# Autodesk Inventor assembly: +XPanel
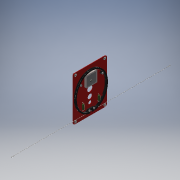
[picture p0: Inventor's stored thumbnail of the model, 180x180]
Saved by Autodesk Inventor 2018 (Build 220112000, 112)
## iProperties
Created: 2018-07-05
Part Number: +XPanel
Document SubType Name: Assembly
Designer: Bradley
Mass: 19.8214 g
Surface Area: 182.188 cm^2
Volume: 10.2774 cm^3
Density: 1.92865 g/cm^3
Author: Bradley
## Documents named in this file (10)
- D:\Users\Bradley\Documents\CougsInSpace\CougSat1-Hardware\CougSat1-AvionicBoard\CADModel\Native\+XPanel.iam
- D:\Users\Bradley\Documents\CougsInSpace\CougSat1-Hardware\CougSat1-AvionicBoard\CADModel\Native\+XPanel_PCB.ipt
- D:\Users\Bradley\Documents\CougsInSpace\Resources\ComponentModels\Electronics\Antenna_GPSPatch.ipt
- D:\Users\Bradley\Documents\CougsInSpace\Resources\ComponentModels\Fasteners\Bolt_M3x0.35_5mm_BH.ipt
- D:\Users\Bradley\Documents\CougsInSpace\CougSat1-Hardware\CougSat1-AvionicBoard\CADModel\Native\+XPanel_AntennaDeployed.ipt
- D:\Users\Bradley\Documents\CougsInSpace\CougSat1-Hardware\CougSat1-AvionicBoard\CADModel\Native\+XPanel_AntennaMount.ipt
- D:\Users\Bradley\Documents\CougsInSpace\CougSat1-Hardware\CougSat1-AvionicBoard\CADModel\Native\+XPanel_AntennaForm.ipt
- D:\Users\Bradley\Documents\CougsInSpace\Resources\ComponentModels\Fasteners\Bolt_M2x0.4_6mm_SH.ipt
- D:\Users\Bradley\Documents\CougsInSpace\CougSat1-Hardware\CougSat1-AvionicBoard\CADModel\Native\+XPanel_AntennaStowed+Y.ipt
- D:\Users\Bradley\Documents\CougsInSpace\Resources\ComponentModels\Electronics\Resistor_TH-15mm.ipt
## Components (17 placed, 9 different names)
1. +XPanel_PCB:1 — Insert:1, Insert:2, Insert:3, Insert:4, Insert:5, Mate:2, Mate:3, Insert:10, Insert:11, Insert:14, Insert:15, Insert:20, Insert:21, Insert:22, Insert:23
2. Antenna_GPSPatch:1 — Flush:1, Insert:1
3. Bolt_M3x0.35_5mm_BH:1 — Insert:2
4. Bolt_M3x0.35_5mm_BH:2 — Insert:3
5. Bolt_M3x0.35_5mm_BH:3 — Insert:4
6. Bolt_M3x0.35_5mm_BH:4 — Insert:5
7. +XPanel_AntennaDeployed:1 — Mate:1, Mate:2, Flush:2
8. +XPanel_AntennaDeployed:2 — Mate:3, Mate:4
9. +XPanel_AntennaMount:1 — Mate:1, Mate:4, Insert:16, Insert:17, Insert:18, Insert:19
10. +XPanel_AntennaForm:1 — Insert:10, Insert:11, Insert:12, Insert:13, Insert:14, Insert:15, Insert:16, Insert:17, Mate:5
11. Bolt_M2x0.4_6mm_SH:1 — Insert:12
12. Bolt_M2x0.4_6mm_SH:2 — Insert:13
13. Bolt_M2x0.4_6mm_SH:3 — Insert:19
14. Bolt_M2x0.4_6mm_SH:4 — Insert:18
15. +XPanel_AntennaStowed+Y:1 — Mate:5, Flush:2
16. Resistor_TH-15mm:1 — Insert:20, Insert:21
17. Resistor_TH-15mm:2 — Insert:22, Insert:23
## Relationships (26: Insert 19, Mate 5, Flush 2)
- Flush:1: Antenna_GPSPatch:1
- Insert:1: +XPanel_PCB:1 ↔ Antenna_GPSPatch:1
- Insert:2: +XPanel_PCB:1 ↔ Bolt_M3x0.35_5mm_BH:1
- Insert:3: +XPanel_PCB:1 ↔ Bolt_M3x0.35_5mm_BH:2
- Insert:4: +XPanel_PCB:1 ↔ Bolt_M3x0.35_5mm_BH:3
- Insert:5: +XPanel_PCB:1 ↔ Bolt_M3x0.35_5mm_BH:4
- Mate:1: +XPanel_AntennaDeployed:1 ↔ +XPanel_AntennaMount:1
- Mate:2: +XPanel_PCB:1 ↔ +XPanel_AntennaDeployed:1
- Mate:3: +XPanel_PCB:1 ↔ +XPanel_AntennaDeployed:2
- Mate:4: +XPanel_AntennaDeployed:2 ↔ +XPanel_AntennaMount:1
- Insert:10: +XPanel_PCB:1 ↔ +XPanel_AntennaForm:1
- Insert:11: +XPanel_PCB:1 ↔ +XPanel_AntennaForm:1
- Insert:12: +XPanel_AntennaForm:1 ↔ Bolt_M2x0.4_6mm_SH:1
- Insert:13: +XPanel_AntennaForm:1 ↔ Bolt_M2x0.4_6mm_SH:2
- Insert:14: +XPanel_PCB:1 ↔ +XPanel_AntennaForm:1
- Insert:15: +XPanel_PCB:1 ↔ +XPanel_AntennaForm:1
- Insert:16: +XPanel_AntennaMount:1 ↔ +XPanel_AntennaForm:1
- Insert:17: +XPanel_AntennaMount:1 ↔ +XPanel_AntennaForm:1
- Insert:18: +XPanel_AntennaMount:1 ↔ Bolt_M2x0.4_6mm_SH:4
- Insert:19: +XPanel_AntennaMount:1 ↔ Bolt_M2x0.4_6mm_SH:3
- Mate:5: +XPanel_AntennaForm:1 ↔ +XPanel_AntennaStowed+Y:1
- Flush:2: +XPanel_AntennaDeployed:1 ↔ +XPanel_AntennaStowed+Y:1
- Insert:20 (-1.2 mm): +XPanel_PCB:1 ↔ Resistor_TH-15mm:1
- Insert:21 (-1.2 mm): +XPanel_PCB:1 ↔ Resistor_TH-15mm:1
- Insert:22 (-1.2 mm): +XPanel_PCB:1 ↔ Resistor_TH-15mm:2
- Insert:23 (-1.2 mm): +XPanel_PCB:1 ↔ Resistor_TH-15mm:2
